# Autodesk Inventor assembly: СтойкаКруглая
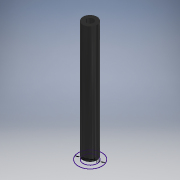
[picture p0: Inventor's stored thumbnail of the model, 180x180]
Saved by Autodesk Inventor 2020 (Build 240168000, 168)
## iProperties
Created: 2025-01-12
Part Number: СтойкаКруглая
Document SubType Name: Assembly
Designer: Ivan
Mass: 15 g
Surface Area: 14.3846 cm^2
Volume: 1.49487 cm^3
Density: 10.0343 g/cm^3
Author: Ivan
## Documents named in this file (3)
- C:\!projects\DASH-\3D\Dash-V1\step\m3_bolt\СтойкаКруглая.iam
- C:\!projects\DASH-\3D\Dash-V1\step\m3_bolt\Spacer Bolts_m3_bn_L5.ipt
- C:\!projects\DASH-\3D\Деталь3.ipt
## Components (3 placed, 2 different names)
1. Spacer Bolts_m3_bn_L5:1 — Совмещение:1, Совмещение:2, Совмещение:3, Угол:1, Угол:2
2. Spacer Bolts_m3_bn_L5:2 — Заподлицо:2, Совмещение:3, Угол:1
3. Деталь3:1 — Заподлицо:3
## Relationships (8: Mate 3, Flush 3, Angle 2)
- Совмещение:1 [Mate]: Spacer Bolts_m3_bn_L5:1
- Совмещение:2 [Mate]: Spacer Bolts_m3_bn_L5:1
- Заподлицо:1 [Flush] (50 mm)
- Заподлицо:2 [Flush]: Spacer Bolts_m3_bn_L5:2
- Совмещение:3 [Mate]: Spacer Bolts_m3_bn_L5:1 ↔ Spacer Bolts_m3_bn_L5:2
- Угол:1 [Angle] (0 deg): Spacer Bolts_m3_bn_L5:1 ↔ Spacer Bolts_m3_bn_L5:2
- Угол:2 [Angle] (0 deg): Spacer Bolts_m3_bn_L5:1
- Заподлицо:3 [Flush]: Деталь3:1
